# Autodesk Inventor assembly: ASY NDM-VOS_powder_hopper
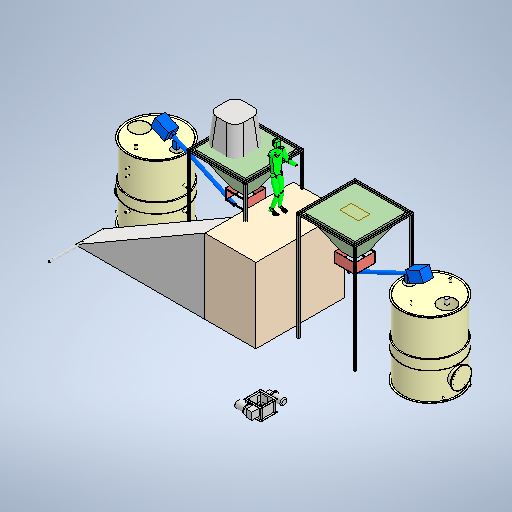
[picture p0: Inventor's stored thumbnail of the model, 512x512]
Saved by Autodesk Inventor 2025 (Build 290162010, 162A)
## iProperties
Created: 2024-07-24
Part Number: ASY NDM-VOS_powder_hopper
Document SubType Name: Assembly
Designer: admin
Author: admin
## Documents named in this file (14)
- C:\Users\pokla\Documents\Inventor\NDM-VOS_powder_hopper\ASY NDM-VOS_powder_hopper.iam
- C:\Users\pokla\Documents\Inventor\NDM-VOS_powder_hopper\Dummy 3.ipt
- C:\Users\pokla\Documents\Inventor\NDM-VOS_powder_hopper\NDM-VOS dummy2.ipt
- C:\Users\pokla\Documents\Inventor\NDM-VOS_powder_hopper\human 01\ч ASY human dummy 01.iam
- C:\Users\pokla\Documents\Inventor\NDM-VOS_powder_hopper\NDM-VOS dummy3.ipt
- C:\Users\pokla\Documents\Inventor\NDM-VOS_powder_hopper\Рама.iam
- C:\Users\pokla\Documents\Inventor\NDM-VOS_powder_hopper\NDM-VOS dummy4.ipt
- C:\Users\pokla\Documents\Inventor\NDM-VOS_powder_hopper\NDM-VOS dummy5.ipt
- C:\Users\pokla\Documents\Inventor\NDM-VOS_powder_hopper\NDM-VOS dummy6.ipt
- C:\Users\pokla\Documents\Inventor\NDM-VOS_powder_hopper\NDM-VOS dummy FLOOR.ipt
- C:\Users\pokla\Documents\Inventor\NDM-VOS_powder_hopper\NDM-VOS dummy Crane.ipt
- C:\Users\pokla\Documents\Inventor\NDM-VOS_powder_hopper\NDM-VOS dummy staircase.ipt
- C:\Users\pokla\Documents\Inventor\NDM-VOS_powder_hopper\NDM-VOS dummy upstairse.ipt
- C:\Users\pokla\Documents\Inventor\NDM-VOS_powder_hopper\Измельчитель комков.ipt
## Components (20 placed, 13 different names)
1. NDM-VOS dummy3:1 — Rotational:1, Mate:5, Mate:9
2. Dummy 3:1 — Flush:1
3. NDM-VOS dummy2:1 — Flush:8, Mate:2, Mate:13, Flush:13, Rigid:2
4. NDM-VOS dummy3:2 — Mate:6, Mate:8, Mate:9, Mate:13, Flush:15
5. Рама:1 [sub-assembly] — Mate:1, Flush:8, Mate:2, Mate:11, Flush:11, Flush:12, Mate:12, Flush:13
6. NDM-VOS dummy4:1
7. NDM-VOS dummy4:2 — Rotational:1
8. NDM-VOS dummy5:2 — Mate:14, Flush:16
9. NDM-VOS dummy5:1 — Flush:9, Flush:15, Mate:14
10. ч ASY human dummy 01:1 [sub-assembly] — Mate:16
11. NDM-VOS dummy6:1 — Rigid:1
12. NDM-VOS dummy2:2 — Flush:14, Rigid:1
13. Рама:2 [sub-assembly] — Mate:11, Flush:11, Flush:12, Flush:14, Flush:18
14. NDM-VOS dummy4:3
15. NDM-VOS dummy6:2 — Rigid:2
16. NDM-VOS dummy FLOOR:1 — Mate:5, Mate:6, Mate:8, Mate:10, Mate:12, Flush:16, Mate:15, Mate:18
17. NDM-VOS dummy Crane:1 — Mate:10
18. NDM-VOS dummy staircase:1 — Mate:15, Mate:16, Mate:17, Flush:17, Flush:18
19. NDM-VOS dummy upstairse:1 — Mate:17, Mate:18, Flush:17
20. Измельчитель комков:1
## Relationships (31: Mate 16, Flush 12, WeldJoint 2, RevoluteJoint 1)
- Flush:1: Dummy 3:1
- Mate:1: Рама:1
- Flush:8: NDM-VOS dummy2:1 ↔ Рама:1
- Mate:2: NDM-VOS dummy2:1 ↔ Рама:1
- Rotational:1 [RevoluteJoint]: NDM-VOS dummy3:1 ↔ NDM-VOS dummy4:2
- Flush:9: NDM-VOS dummy5:1
- [Flush]: NDM-VOS dummy2:2 ↔ Рама:2
- [Mate]: NDM-VOS dummy2:2 ↔ Рама:2
- Mate:5: NDM-VOS dummy3:1 ↔ NDM-VOS dummy FLOOR:1
- Mate:6: NDM-VOS dummy3:2 ↔ NDM-VOS dummy FLOOR:1
- Mate:8 (1200 mm): NDM-VOS dummy3:2 ↔ NDM-VOS dummy FLOOR:1
- Mate:9 (-1830 mm): NDM-VOS dummy3:1 ↔ NDM-VOS dummy3:2
- Mate:10 (3500 mm): NDM-VOS dummy FLOOR:1 ↔ NDM-VOS dummy Crane:1
- Mate:11 (1500 mm): Рама:1 ↔ Рама:2
- Flush:11: Рама:1 ↔ Рама:2
- Flush:12: Рама:1 ↔ Рама:2
- Mate:12: Рама:1 ↔ NDM-VOS dummy FLOOR:1
- Mate:13: NDM-VOS dummy2:1 ↔ NDM-VOS dummy3:2
- Flush:13: NDM-VOS dummy2:1 ↔ Рама:1
- Flush:14: NDM-VOS dummy2:2 ↔ Рама:2
- Flush:15: NDM-VOS dummy3:2 ↔ NDM-VOS dummy5:1
- Rigid:1 [WeldJoint]: NDM-VOS dummy6:1 ↔ NDM-VOS dummy2:2
- Rigid:2 [WeldJoint]: NDM-VOS dummy2:1 ↔ NDM-VOS dummy6:2
- Mate:14: NDM-VOS dummy5:2 ↔ NDM-VOS dummy5:1
- Flush:16: NDM-VOS dummy5:2 ↔ NDM-VOS dummy FLOOR:1
- Mate:15: NDM-VOS dummy FLOOR:1 ↔ NDM-VOS dummy staircase:1
- Mate:16: ч ASY human dummy 01:1 ↔ NDM-VOS dummy staircase:1
- Mate:17: NDM-VOS dummy staircase:1 ↔ NDM-VOS dummy upstairse:1
- Mate:18: NDM-VOS dummy FLOOR:1 ↔ NDM-VOS dummy upstairse:1
- Flush:17: NDM-VOS dummy staircase:1 ↔ NDM-VOS dummy upstairse:1
- Flush:18: Рама:2 ↔ NDM-VOS dummy staircase:1
## Named parameters: d20_d12 = 0 mm, d21_d13 = 0 mm
